# Autodesk Inventor assembly: SpoolWinder
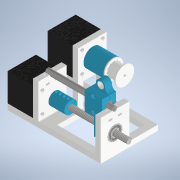
[picture p0: Inventor's stored thumbnail of the model, 180x180]
Saved by Autodesk Inventor 2021 (Build 250183000, 183)
## iProperties
Created: 2021-03-11
Part Number: SpoolWinder
Document SubType Name: Assembly
Designer: elmar
Author: elmar
## Documents named in this file (15)
- D:\MyRepos\SpoolRewinder\SpoolWinder.iam
- D:\MyRepos\SpoolRewinder\CableGuide.ipt
- D:\MyRepos\SpoolRewinder\WinderBase.ipt
- D:\MyRepos\SpoolRewinder\DestinationSpoolHolder.ipt
- C:\Users\elmar\OneDrive\Documents\Inventor\Content Center Files\R2021\en-US\Bearing GB_T 292-2007\Rolling bearing B708 C GB_T 292-2007.ipt
- C:\Users\elmar\OneDrive\Documents\Inventor\Content Center Files\R2021\en-US\Bearing GB_T 16940\Linear motion bearing LBP 81524 GB_T 16940.ipt
- D:\MyRepos\SpoolRewinder\8mmx100mmShaft.ipt
- D:\MyRepos\SpoolRewinder\ACMET8x100mmShaft.ipt
- D:\MyRepos\SpoolRewinder\NEMA17.ipt
- D:\MyRepos\SpoolRewinder\NEMA17toACMETr8.ipt
- D:\MyRepos\SpoolRewinder\Spool.ipt
- D:\MyRepos\SpoolRewinder\CableGuideInsert.ipt
- D:\MyRepos\SpoolRewinder\Arduino UNO R3.ipt
- D:\MyRepos\SpoolRewinder\L298N Dual H Bridge.ipt
- D:\MyRepos\SpoolRewinder\ElectronicsPlate.ipt
## Components (16 placed, 14 different names)
1. CableGuide:1 — Insert:4, Mate:7, Insert:9, Mate:9
2. WinderBase:1 — Mate:1, Insert:3, Insert:5, Mate:7, Insert:10, Angle:1, Insert:16, Insert:17
3. DestinationSpoolHolder:1 — Insert:3, Insert:8
4. Bearing GB/T 292-2007 Type IN - withdrawn B708 C:1 — Insert:10
5. Bearing GB/T 16940 LBP 81524:1 — Insert:4, Mate:3
6. 8mmx100mmShaft:1 — Insert:5, Mate:3
7. ACMET8x100mmShaft:1 — Mate:6, Mate:8, Mate:9
8. NEMA17:1 — Mate:1, Mate:6, Insert:7, Insert:17
9. NEMA17:2 — Angle:1, Insert:16
10. NEMA17toACMETr8:1 — Insert:7, Mate:8
11. Spool:1 — Insert:8
12. CableGuideInsert:1 — Insert:9
13. Arduino UNO R3:1 — Insert:11
14. L298N Dual H Bridge:1 — Insert:12, Insert:15
15. L298N Dual H Bridge:2 — Insert:13, Insert:14
16. ElectronicsPlate:1 — Insert:11, Insert:12, Insert:13, Insert:14, Insert:15
## Relationships (21: Insert 14, Mate 6, Angle 1)
- Mate:1: WinderBase:1 ↔ NEMA17:1
- Insert:3 (1 mm): WinderBase:1 ↔ DestinationSpoolHolder:1
- Insert:4: CableGuide:1 ↔ Bearing GB/T 16940 LBP 81524:1
- Insert:5 (1 mm): WinderBase:1 ↔ 8mmx100mmShaft:1
- Mate:3: Bearing GB/T 16940 LBP 81524:1 ↔ 8mmx100mmShaft:1
- Mate:6: ACMET8x100mmShaft:1 ↔ NEMA17:1
- Mate:7 (1 mm): CableGuide:1 ↔ WinderBase:1
- Insert:7 (-12 mm): NEMA17:1 ↔ NEMA17toACMETr8:1
- Insert:8: DestinationSpoolHolder:1 ↔ Spool:1
- Insert:9: CableGuide:1 ↔ CableGuideInsert:1
- Insert:10: WinderBase:1 ↔ Bearing GB/T 292-2007 Type IN - withdrawn B708 C:1
- Mate:8: ACMET8x100mmShaft:1 ↔ NEMA17toACMETr8:1
- Mate:9: CableGuide:1 ↔ ACMET8x100mmShaft:1
- Insert:11: Arduino UNO R3:1 ↔ ElectronicsPlate:1
- Insert:12: L298N Dual H Bridge:1 ↔ ElectronicsPlate:1
- Insert:13: L298N Dual H Bridge:2 ↔ ElectronicsPlate:1
- Insert:14: L298N Dual H Bridge:2 ↔ ElectronicsPlate:1
- Insert:15: L298N Dual H Bridge:1 ↔ ElectronicsPlate:1
- Angle:1 (0 deg): WinderBase:1 ↔ NEMA17:2
- Insert:16: WinderBase:1 ↔ NEMA17:2
- Insert:17: WinderBase:1 ↔ NEMA17:1
